# Autodesk Inventor assembly: geared_wheels
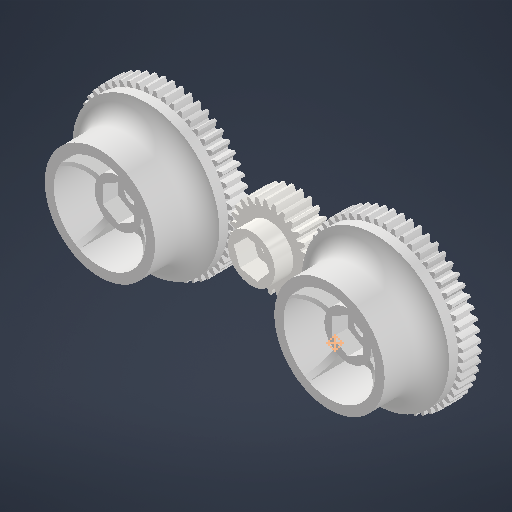
[picture p0: Inventor's stored thumbnail of the model, 512x512]
Saved by Autodesk Inventor 2027.1 (Build 311270010, 270A)
## iProperties
Created: 2026-10-03
Part Number: geared_wheels
Document SubType Name: Assembly
Designer: ajrcr
Author: ajrcr
## Documents named in this file (3)
- C:\Users\ajrcr\OneDrive\Documents\Y3_s2\MCTR327\Git_Repo\Design-2026\3D parts\geared_wheels.iam
- C:\Users\ajrcr\OneDrive\Documents\Y3_s2\MCTR327\Git_Repo\Design-2026\3D parts\wheel_v4.ipt
- C:\Users\ajrcr\OneDrive\Documents\Y3_s2\MCTR327\Git_Repo\Design-2026\3D parts\geared_wheels\Design Accelerator\Spur Gears1.iam
## Components (3 placed, 2 different names)
1. wheel_v4:1 — Mate:1, Flush:1
2. Spur Gears:1 [sub-assembly] — Mate:1, Mate:2, Flush:1, Flush:2
3. wheel_v4:2 — Mate:2, Flush:2
## Relationships (4: Mate 2, Flush 2)
- Mate:1 (62.5 mm): wheel_v4:1 ↔ Spur Gears:1
- Mate:2 (62.5 mm): Spur Gears:1 ↔ wheel_v4:2
- Flush:1: wheel_v4:1 ↔ Spur Gears:1
- Flush:2: Spur Gears:1 ↔ wheel_v4:2
